# Autodesk Inventor assembly: 20220523_仮機体
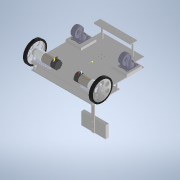
[picture p0: Inventor's stored thumbnail of the model, 180x180]
Saved by Autodesk Inventor 2020 (Build 240168000, 168)
## iProperties
Created: 2022-05-22
Part Number: 20220523_仮機体
Document SubType Name: Assembly
Designer: Naggy
Author: Naggy
## Documents named in this file (15)
- C:\Users\Naggy\Documents\Inventor\robot_design2020\20220523_仮機体.iam
- C:\Users\Naggy\Documents\Inventor\robot_design2020\20220522.ipt
- C:\Users\Naggy\Documents\Inventor\robot_design2020\20220509_知能ロボットキャスタ.ipt
- C:\Users\Naggy\Documents\Inventor\robot_design2020\20220519モータを取り付けるやつ.ipt
- C:\Users\Naggy\Documents\Inventor\robot_design2020\20220519知能ロボットモータとエンコーダ.ipt
- C:\Users\Naggy\Documents\Inventor\robot_design2020\RD003_キャスタ420G-R32 (3).ipt
- C:\Users\Naggy\Documents\Inventor\robot_design2020\20220508_知能ロボットスペーサ.ipt
- C:\Users\Naggy\Documents\Inventor\robot_design2020\20220523_知能ロボット2階部分.ipt
- C:\Users\Naggy\Documents\Inventor\robot_design2020\20220509_知能ロボットカメラ土台.ipt
- C:\Users\Naggy\Documents\Inventor\robot_design2020\20220523_センサモジュール.ipt
- C:\Users\Naggy\Documents\Inventor\robot_design2020\20220523_スペーサ.ipt
- C:\Users\Naggy\Documents\Inventor\robot_design2020\20220524_70アルミホイール.ipt
- C:\Users\Naggy\Documents\Inventor\robot_design2020\20220524_知能ロボットカメラ固定部品.ipt
- C:\Users\Naggy\Documents\Inventor\robot_design2020\20220524_仮サーボ.iam
- C:\Users\Naggy\Documents\Inventor\robot_design2020\20220523_吸引部分.ipt
## Components (23 placed, 14 different names)
1. 20220522:1 — メイト:3, メイト:4, メイト:9, メイト:10, メイト:13, メイト:14, メイト:15, メイト:16, メイト:21, メイト:22, メイト:27, メイト:29
2. 20220519モータを取り付けるやつ:2 — メイト:4, メイト:5
3. 20220519モータを取り付けるやつ:3 — メイト:3, メイト:6
4. 20220519知能ロボットモータとエンコーダ:1 — メイト:5, メイト:25
5. 20220519知能ロボットモータとエンコーダ:2 — メイト:6, メイト:26
6. 20220509_知能ロボットキャスタ:3 — メイト:9, メイト:11
7. RD003_キャスタ420G-R32 (3):3 — メイト:11
8. RD003_キャスタ420G-R32 (3):4 — メイト:12
9. 20220509_知能ロボットキャスタ:4 — メイト:10, メイト:12
10. 20220508_知能ロボットスペーサ:1 — メイト:14
11. 20220508_知能ロボットスペーサ:2 — メイト:16
12. 20220508_知能ロボットスペーサ:3 — メイト:13, メイト:17
13. 20220508_知能ロボットスペーサ:4 — メイト:15
14. 20220523_知能ロボット2階部分:1 — メイト:17
15. 20220523_センサモジュール:1 — メイト:23, メイト:24
16. 20220523_スペーサ:1 — メイト:21, メイト:23, メイト:24
17. 20220523_スペーサ:2 — メイト:22
18. 20220524_70アルミホイール:1 — メイト:26
19. 20220524_70アルミホイール:4 — メイト:25
20. 20220524_知能ロボットカメラ固定部品:1 — メイト:27, メイト:28
21. 20220509_知能ロボットカメラ土台:1 — メイト:28
22. 20220524_仮サーボ:1 [sub-assembly] — メイト:29, メイト:30
23. 20220523_吸引部分:1 — メイト:30
## Relationships (23: Mate 23)
- メイト:3 [Mate]: 20220522:1 ↔ 20220519モータを取り付けるやつ:3
- メイト:4 [Mate]: 20220522:1 ↔ 20220519モータを取り付けるやつ:2
- メイト:5 [Mate]: 20220519モータを取り付けるやつ:2 ↔ 20220519知能ロボットモータとエンコーダ:1
- メイト:6 [Mate]: 20220519モータを取り付けるやつ:3 ↔ 20220519知能ロボットモータとエンコーダ:2
- メイト:9 [Mate]: 20220522:1 ↔ 20220509_知能ロボットキャスタ:3
- メイト:10 [Mate]: 20220522:1 ↔ 20220509_知能ロボットキャスタ:4
- メイト:11 [Mate]: 20220509_知能ロボットキャスタ:3 ↔ RD003_キャスタ420G-R32 (3):3
- メイト:12 [Mate]: RD003_キャスタ420G-R32 (3):4 ↔ 20220509_知能ロボットキャスタ:4
- メイト:13 [Mate]: 20220522:1 ↔ 20220508_知能ロボットスペーサ:3
- メイト:14 [Mate]: 20220522:1 ↔ 20220508_知能ロボットスペーサ:1
- メイト:15 [Mate]: 20220522:1 ↔ 20220508_知能ロボットスペーサ:4
- メイト:16 [Mate]: 20220522:1 ↔ 20220508_知能ロボットスペーサ:2
- メイト:17 [Mate]: 20220508_知能ロボットスペーサ:3 ↔ 20220523_知能ロボット2階部分:1
- メイト:21 [Mate]: 20220522:1 ↔ 20220523_スペーサ:1
- メイト:22 [Mate]: 20220522:1 ↔ 20220523_スペーサ:2
- メイト:23 [Mate]: 20220523_センサモジュール:1 ↔ 20220523_スペーサ:1
- メイト:24 [Mate]: 20220523_センサモジュール:1 ↔ 20220523_スペーサ:1
- メイト:25 [Mate]: 20220519知能ロボットモータとエンコーダ:1 ↔ 20220524_70アルミホイール:4
- メイト:26 [Mate]: 20220519知能ロボットモータとエンコーダ:2 ↔ 20220524_70アルミホイール:1
- メイト:27 [Mate]: 20220522:1 ↔ 20220524_知能ロボットカメラ固定部品:1
- メイト:28 [Mate]: 20220524_知能ロボットカメラ固定部品:1 ↔ 20220509_知能ロボットカメラ土台:1
- メイト:29 [Mate]: 20220522:1 ↔ 20220524_仮サーボ:1
- メイト:30 [Mate]: 20220524_仮サーボ:1 ↔ 20220523_吸引部分:1
